# Autodesk Inventor assembly: 1x2 Terminal Block
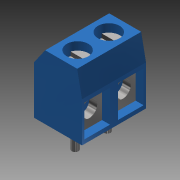
[picture p0: Inventor's stored thumbnail of the model, 180x180]
Saved by Autodesk Inventor 2013 (Build 170138000, 138)
## iProperties
Created: 2014-12-22
Part Number: 1x2 Terminal Block
Document SubType Name: Assembly
Designer: Kyle
Author: Kyle
## Documents named in this file (5)
- C:\Users\Kyle\Documents\Autodesk\Output\Inventor 2013\Electronics\Terminals\1x2 Terminal Block.iam
- C:\Users\Kyle\Documents\Autodesk\Output\Inventor 2013\Electronics\Sub-Components\Multipieces\1x2 Terminal Block Body.ipt
- C:\Users\Kyle\Documents\Autodesk\Output\Inventor 2013\Electronics\Sub-Components\Multipieces\Terminal Block Screw.ipt
- C:\Users\Kyle\Documents\Autodesk\Output\Inventor 2013\Electronics\Sub-Components\Multipieces\Terminal Block Terminal.ipt
- C:\Users\Kyle\Documents\Autodesk\Output\Inventor 2013\Electronics\Sub-Components\Leads\0.15 Lead.ipt
## Components (7 placed, 4 different names)
1. 1x2 Terminal Block Body:1 — Mate:1, Mate:2, Mate:3, Mate:4, Mate:5, Mate:6, Mate:7, Mate:8, Mate:9, Mate:10, Mate:11, Mate:12, Mate:14, Mate:15, Mate:16
2. Terminal Block Screw:1 — Mate:1, Mate:2
3. Terminal Block Screw:2 — Mate:3, Mate:4
4. Terminal Block Terminal:1 — Mate:5, Mate:6, Mate:7
5. Terminal Block Terminal:2 — Mate:8, Mate:9, Mate:10
6. 0.15 Lead:1 — Mate:11, Mate:13, Mate:14
7. 0.15 Lead:2 — Mate:12, Mate:13, Mate:15, Mate:16
## Relationships (16: Mate 16)
- Mate:1: 1x2 Terminal Block Body:1 ↔ Terminal Block Screw:1
- Mate:2: 1x2 Terminal Block Body:1 ↔ Terminal Block Screw:1
- Mate:3: 1x2 Terminal Block Body:1 ↔ Terminal Block Screw:2
- Mate:4: 1x2 Terminal Block Body:1 ↔ Terminal Block Screw:2
- Mate:5: 1x2 Terminal Block Body:1 ↔ Terminal Block Terminal:1
- Mate:6: 1x2 Terminal Block Body:1 ↔ Terminal Block Terminal:1
- Mate:7: 1x2 Terminal Block Body:1 ↔ Terminal Block Terminal:1
- Mate:8: 1x2 Terminal Block Body:1 ↔ Terminal Block Terminal:2
- Mate:9: 1x2 Terminal Block Body:1 ↔ Terminal Block Terminal:2
- Mate:10: 1x2 Terminal Block Body:1 ↔ Terminal Block Terminal:2
- Mate:11: 1x2 Terminal Block Body:1 ↔ 0.15 Lead:1
- Mate:12: 1x2 Terminal Block Body:1 ↔ 0.15 Lead:2
- Mate:13 (5.08 mm): 0.15 Lead:1 ↔ 0.15 Lead:2
- Mate:14 (-3.81 mm): 1x2 Terminal Block Body:1 ↔ 0.15 Lead:1
- Mate:15 (-3.81 mm): 1x2 Terminal Block Body:1 ↔ 0.15 Lead:2
- Mate:16 (-2.7305 mm): 1x2 Terminal Block Body:1 ↔ 0.15 Lead:2
